# Autodesk Inventor assembly: Case Top
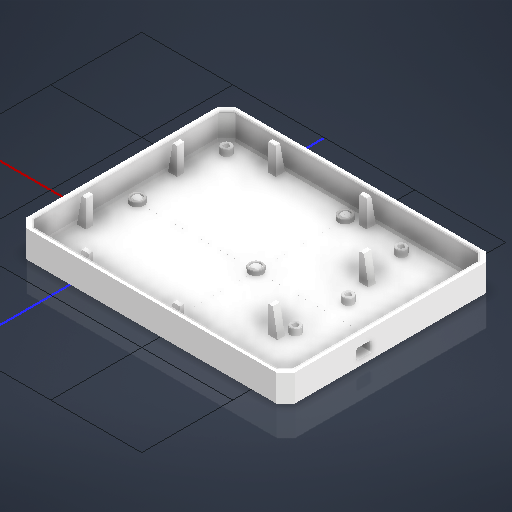
[picture p0: Inventor's stored thumbnail of the model, 512x512]
Saved by Autodesk Inventor 2026 (Build 300175000, 175)
## iProperties
Created: 2025-06-07
Part Number: Case Top
Document SubType Name: Assembly
Designer: ckyiu
Author: ckyiu
## Documents named in this file (6)
- F:\Chessboard-Design\Assemblies\Case\Case Bottom.iam
- F:\Chessboard-Design\Parts\Case\Bottom\Case Bottom Ring.ipt
- F:\Chessboard-Design\Parts\Case\Bottom\Case Bottom TL.ipt
- F:\Chessboard-Design\Parts\Case\Bottom\Case Bottom TR.ipt
- F:\Chessboard-Design\Parts\Case\Bottom\Case Bottom BL.ipt
- F:\Chessboard-Design\Parts\Case\Bottom\Case Bottom BR.ipt
## Components (9 placed, 5 different names)
1. Case Bottom TL:1 — Mate:1, Mate:2, Flush:1, Flush:2, Flush:4, Insert:1
2. Case Bottom TR:1 — Mate:2, Mate:3, Flush:2, Flush:3, Insert:2, Insert:5
3. Case Bottom BL:1 — Mate:1, Mate:4, Flush:1, Flush:4, Flush:5
4. Case Bottom BR:1 — Mate:3, Mate:4, Flush:3, Flush:5, Insert:3, Insert:4
5. Case Bottom Ring:1 — Insert:1
6. Case Bottom Ring:2 — Insert:2
7. Case Bottom Ring:3 — Insert:3
8. Case Bottom Ring:4 — Insert:5
9. Case Bottom Ring:5 — Insert:4
## Relationships (14: Flush 5, Insert 5, Mate 4)
- Mate:1: Case Bottom TL:1 ↔ Case Bottom BL:1
- Mate:2: Case Bottom TL:1 ↔ Case Bottom TR:1
- Mate:3: Case Bottom TR:1 ↔ Case Bottom BR:1
- Mate:4: Case Bottom BL:1 ↔ Case Bottom BR:1
- Flush:1: Case Bottom TL:1 ↔ Case Bottom BL:1
- Flush:2: Case Bottom TL:1 ↔ Case Bottom TR:1
- Flush:3: Case Bottom TR:1 ↔ Case Bottom BR:1
- Flush:4: Case Bottom TL:1 ↔ Case Bottom BL:1
- Flush:5: Case Bottom BL:1 ↔ Case Bottom BR:1
- Insert:1: Case Bottom TL:1 ↔ Case Bottom Ring:1
- Insert:2: Case Bottom TR:1 ↔ Case Bottom Ring:2
- Insert:3: Case Bottom BR:1 ↔ Case Bottom Ring:3
- Insert:4: Case Bottom BR:1 ↔ Case Bottom Ring:5
- Insert:5: Case Bottom TR:1 ↔ Case Bottom Ring:4
